# Autodesk Inventor assembly: !SCARA assembly
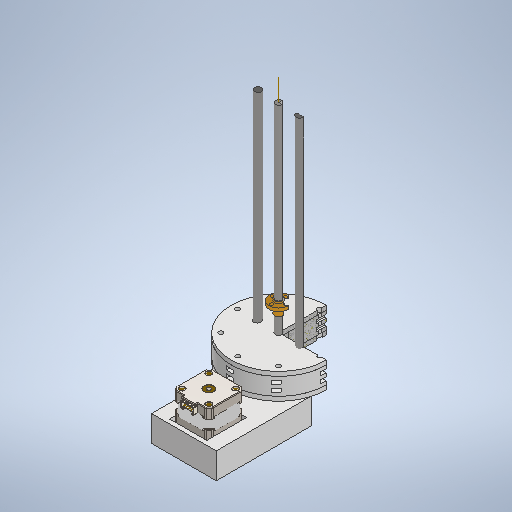
[picture p0: Inventor's stored thumbnail of the model, 512x512]
Saved by Autodesk Inventor 2025.2 (Build 292293000, 293)
## iProperties
Created: 2025-01-25
Part Number: !SCARA assembly
Document SubType Name: Assembly
Designer: caomi
Author: caomi
## Documents named in this file (11)
- C:\Minh Nguyen\H2A\cad\SCARA\!SCARA assembly.iam
- C:\Minh Nguyen\H2A\cad\SCARA\SCARA base.ipt
- C:\Minh Nguyen\H2A\cad\SCARA\Stepper Motor 17HS3401.ipt
- C:\Minh Nguyen\H2A\cad\SCARA\608 Bearing.ipt
- C:\Minh Nguyen\H2A\cad\SCARA\SCARA swivel base - top.ipt
- C:\Minh Nguyen\H2A\cad\SCARA\Shaft support.ipt
- C:\Minh Nguyen\H2A\cad\SCARA\SCARA swivel base - bottom.ipt
- C:\Minh Nguyen\H2A\cad\SCARA\Guide rods.ipt
- C:\Minh Nguyen\H2A\cad\SCARA\SCARA swivel base - mid.ipt
- C:\Minh Nguyen\H2A\cad\SCARA\Lead screw.ipt
- C:\Minh Nguyen\H2A\cad\SCARA\SCARA swivel connection rod.ipt
## Components (13 placed, 10 different names)
1. SCARA base:1 — Slider:2, Rigid:1, Rotational:1
2. Stepper Motor 17HS3401:1 — Slider:2
3. 608 Bearing:1 — Rigid:1
4. SCARA swivel base - bottom:1 — Rotational:1, Rigid:2
5. SCARA swivel base - mid:1 — Rigid:2, Rigid:3, Rigid:4, Rigid:5, Rotational:2, Rigid:9
6. Shaft support:1 — Rigid:4, Rigid:7
7. Shaft support:2 — Rigid:3, Rigid:6
8. 608 Bearing:2 — Rigid:5, Rigid:8
9. SCARA swivel base - top:1 — Rotational:2
10. Guide rods:1 — Rigid:6
11. Guide rods:2 — Rigid:7
12. Lead screw:1 — Rigid:8
13. SCARA swivel connection rod:1 — Rigid:9
## Relationships (12: WeldJoint 9, RevoluteJoint 2, TranslationJoint 1)
- Slider:2 [TranslationJoint]: SCARA base:1 ↔ Stepper Motor 17HS3401:1
- Rigid:1 [WeldJoint]: SCARA base:1 ↔ 608 Bearing:1
- Rotational:1 [RevoluteJoint]: SCARA base:1 ↔ SCARA swivel base - bottom:1
- Rigid:2 [WeldJoint]: SCARA swivel base - bottom:1 ↔ SCARA swivel base - mid:1
- Rigid:3 [WeldJoint]: SCARA swivel base - mid:1 ↔ Shaft support:2
- Rigid:4 [WeldJoint]: SCARA swivel base - mid:1 ↔ Shaft support:1
- Rigid:5 [WeldJoint]: SCARA swivel base - mid:1 ↔ 608 Bearing:2
- Rotational:2 [RevoluteJoint]: SCARA swivel base - mid:1 ↔ SCARA swivel base - top:1
- Rigid:6 [WeldJoint]: Shaft support:2 ↔ Guide rods:1
- Rigid:7 [WeldJoint]: Shaft support:1 ↔ Guide rods:2
- Rigid:8 [WeldJoint]: 608 Bearing:2 ↔ Lead screw:1
- Rigid:9 [WeldJoint]: SCARA swivel base - mid:1 ↔ SCARA swivel connection rod:1
